# Autodesk Inventor assembly: A1-19027-300-00 Spool RD-235-2-D-2-1
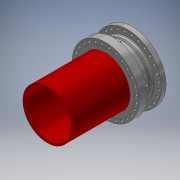
[picture p0: Inventor's stored thumbnail of the model, 180x180]
Saved by Autodesk Inventor 2017.3 (Build 213257000, 257)
## iProperties
Created: 2019-09-12
Part Number: A1-19027-300-00 Spool RD-235-2-D-2-1
Document SubType Name: Weldment
Designer: GVD
Weld Material: Steel, Mild, Welded
Mass: 1.26391e+06 g
Surface Area: 113889 cm^2
Volume: 166321 cm^3
Density: 7.59922 g/cm^3
Author: GVD
## Documents named in this file (7)
- N:\A1 - Projects\A1-19\A1-19027--Syncrude Aurora HT2 spools - SP-237\A1-19027-300-00 Spool RD-235-2-D-2-1.iam
- N:\A1 - Projects\A1-19\A1-19027--Syncrude Aurora HT2 spools - SP-237\A1-19027-300-01 32in pipe.ipt
- N:\A1 - Projects\A1-19\A1-19027--Syncrude Aurora HT2 spools - SP-237\A1-19027-300-02 32in CL150 RF flange.ipt
- N:\A1 - Projects\A1-19\A1-19027--Syncrude Aurora HT2 spools - SP-237\A1-19027-300-04 HCWI liner - nozzle.ipt
- N:\Penticton Foundry\Tag mount - 3in.ipt
- N:\Inventor\Content Center Files\R2017\en-US\ASME B16.11(23)\ASME B16.11 Hex Head Plug 3_4.ipt
- N:\A1 - Projects\A1-19\A1-19027--Syncrude Aurora HT2 spools - SP-237\A1-19027-300-03 32in CL150 FFWN flange.ipt
## Components (8 placed, 6 different names)
1. A1-19027-300-01 32in pipe:1 — Mate:2, Angle:1, Insert:1, Insert:2, Angle:3, Angle:4, Flush:1, Tangent:1, Mate:3, Angle:5, Tangent:2, Angle:6
2. A1-19027-300-02 32in CL150 RF flange:1 — Insert:2, Angle:3
3. A1-19027-300-03 32in CL150 FFWN flange:1 — Mate:1, Insert:1, Insert:3, Flush:2
4. A1-19027-300-04 HCWI liner - nozzle:1 — Insert:3, Angle:4
5. A1-18023-150-08 Tag mount:1 — Flush:1, Flush:2, Tangent:1
6. A1-18023-150-08 Tag mount:2
7. ASME B16.11 Hex Head Plug 3/4:1 — Mate:3, Angle:5, Tangent:2, Angle:6
8. ASME B16.11 Hex Head Plug 3/4:2
## Component patterns: (2 elements, first: A1-18023-150-08 Tag mount:1), (2 elements, first: ASME B16.11 Hex Head Plug 3/4:1)
## Relationships (16: Angle 6, Mate 3, Insert 3, Flush 2, Tangent 2)
- Mate:1: A1-19027-300-03 32in CL150 FFWN flange:1
- Mate:2: A1-19027-300-01 32in pipe:1
- Angle:1 (0 deg): A1-19027-300-01 32in pipe:1
- Insert:1 (2.3813 mm): A1-19027-300-01 32in pipe:1 ↔ A1-19027-300-03 32in CL150 FFWN flange:1
- [Angle] (0 deg): A1-19027-300-01 32in pipe:1 ↔ A1-19027-300-03 32in CL150 FFWN flange:1
- Insert:2 (2.3813 mm): A1-19027-300-01 32in pipe:1 ↔ A1-19027-300-02 32in CL150 RF flange:1
- Angle:3 (0 deg): A1-19027-300-01 32in pipe:1 ↔ A1-19027-300-02 32in CL150 RF flange:1
- Insert:3: A1-19027-300-03 32in CL150 FFWN flange:1 ↔ A1-19027-300-04 HCWI liner - nozzle:1
- Angle:4 (0 deg): A1-19027-300-01 32in pipe:1 ↔ A1-19027-300-04 HCWI liner - nozzle:1
- Flush:1: A1-19027-300-01 32in pipe:1 ↔ A1-18023-150-08 Tag mount:1
- Flush:2 (190.5 mm): A1-19027-300-03 32in CL150 FFWN flange:1 ↔ A1-18023-150-08 Tag mount:1
- Tangent:1: A1-19027-300-01 32in pipe:1 ↔ A1-18023-150-08 Tag mount:1
- Mate:3: A1-19027-300-01 32in pipe:1 ↔ ASME B16.11 Hex Head Plug 3/4:1
- Angle:5 (180 deg): A1-19027-300-01 32in pipe:1 ↔ ASME B16.11 Hex Head Plug 3/4:1
- Tangent:2 (-12.2428 mm): A1-19027-300-01 32in pipe:1 ↔ ASME B16.11 Hex Head Plug 3/4:1
- Angle:6 (0 deg): A1-19027-300-01 32in pipe:1 ↔ ASME B16.11 Hex Head Plug 3/4:1
